# Autodesk Inventor assembly: leg_upper
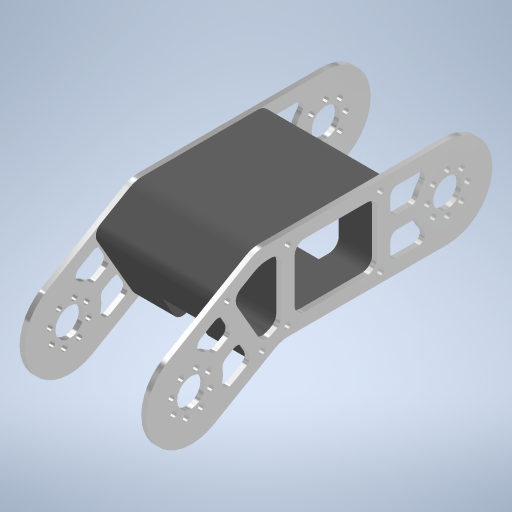
[picture p0: Inventor's stored thumbnail of the model, 512x512]
Saved by Autodesk Inventor 2024.1 (Build 281209000, 209)
## iProperties
Created: 2024-02-11
Part Number: leg_upper
Document SubType Name: Assembly
Designer: hibik
Author: hibik
## Documents named in this file (3)
- C:\Users\hibik\Documents\Robomech\HR\Eglantyne\hard\leg\leg_upper.iam
- C:\Users\hibik\Documents\Robomech\HR\Eglantyne\hard\leg\leg_upper.ipt
- C:\Users\hibik\Documents\Robomech\HR\Eglantyne\hard\leg\leg_upper_middle.ipt
## Components (3 placed, 2 different names)
1. leg_upper:1 — メイト:1, フラッシュ:1, フラッシュ:2, フラッシュ:3, フラッシュ:4, フラッシュ:5
2. leg_upper:2 — メイト:2, フラッシュ:4, フラッシュ:5
3. leg_upper_middle:1 — メイト:1, フラッシュ:1, フラッシュ:2, フラッシュ:3, メイト:2
## Relationships (7: Flush 5, Mate 2)
- メイト:1 [Mate]: leg_upper:1 ↔ leg_upper_middle:1
- フラッシュ:1 [Flush]: leg_upper:1 ↔ leg_upper_middle:1
- フラッシュ:2 [Flush]: leg_upper:1 ↔ leg_upper_middle:1
- フラッシュ:3 [Flush]: leg_upper:1 ↔ leg_upper_middle:1
- メイト:2 [Mate]: leg_upper:2 ↔ leg_upper_middle:1
- フラッシュ:4 [Flush]: leg_upper:1 ↔ leg_upper:2
- フラッシュ:5 [Flush]: leg_upper:1 ↔ leg_upper:2
